# Autodesk Inventor assembly: electronics_assembly
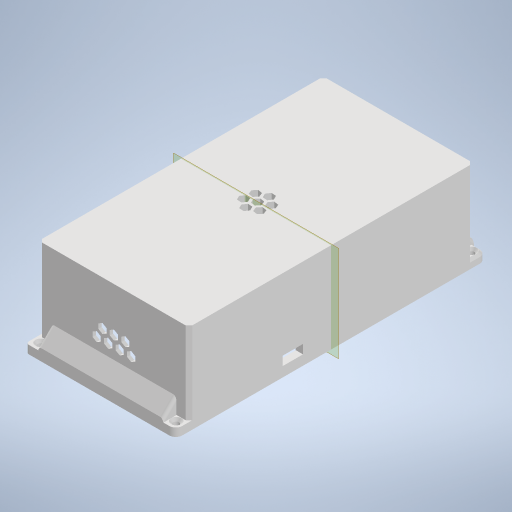
[picture p0: Inventor's stored thumbnail of the model, 512x512]
Saved by Autodesk Inventor 2024.2 (Build 282272000, 272)
## iProperties
Created: 2024-03-06
Part Number: electronics_assembly
Document SubType Name: Assembly
Designer: crow
Author: crow
## Documents named in this file (3)
- C:\Users\crow\Documents\Github\EspFlatPanel\3d_print\inventor_Flat_Panel\electronics_assembly.iam
- C:\Users\crow\Documents\Github\EspFlatPanel\3d_print\inventor_Flat_Panel\electronics-mount.ipt
- C:\Users\crow\Documents\Github\EspFlatPanel\3d_print\inventor_Flat_Panel\battery_holder.ipt
## Components (2 placed, 2 different names)
1. electronics-mount:1 — Rotational:1
2. battery_holder:1 — Rotational:1
## Relationships (1: RevoluteJoint 1)
- Rotational:1 [RevoluteJoint]: electronics-mount:1 ↔ battery_holder:1
